# Autodesk Inventor assembly: krat houder
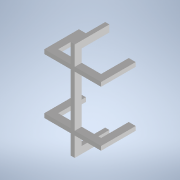
[picture p0: Inventor's stored thumbnail of the model, 180x180]
Saved by Autodesk Inventor 2021 (Build 250183000, 183)
## iProperties
Created: 2022-02-02
Part Number: krat houder
Document SubType Name: Assembly
Designer: ryan
Author: ryan
## Documents named in this file (3)
- C:\Users\ryan\Desktop\git\projecten\school-P2-auto\modellen\inventor\auto moddellen nieuwste\krat houder.iam
- C:\Users\ryan\Desktop\git\projecten\school-P2-auto\modellen\inventor\auto moddellen nieuwste\CONTAINERHOUDER LANG.ipt
- C:\Users\ryan\Desktop\git\projecten\school-P2-auto\modellen\inventor\auto moddellen nieuwste\CONTAINERHOUDER KORT.ipt
## Components (3 placed, 2 different names)
1. CONTAINERHOUDER LANG:1 — Mate:1, Mate:2, Mate:3, Mate:4, Mate:5, Mate:6
2. CONTAINERHOUDER KORT:1 — Mate:1, Mate:4, Mate:5
3. CONTAINERHOUDER KORT:2 — Mate:2, Mate:3, Mate:6
## Relationships (6: Mate 6)
- Mate:1: CONTAINERHOUDER LANG:1 ↔ CONTAINERHOUDER KORT:1
- Mate:2: CONTAINERHOUDER LANG:1 ↔ CONTAINERHOUDER KORT:2
- Mate:3: CONTAINERHOUDER LANG:1 ↔ CONTAINERHOUDER KORT:2
- Mate:4: CONTAINERHOUDER LANG:1 ↔ CONTAINERHOUDER KORT:1
- Mate:5: CONTAINERHOUDER LANG:1 ↔ CONTAINERHOUDER KORT:1
- Mate:6: CONTAINERHOUDER LANG:1 ↔ CONTAINERHOUDER KORT:2
